# Autodesk Inventor assembly: embasev2
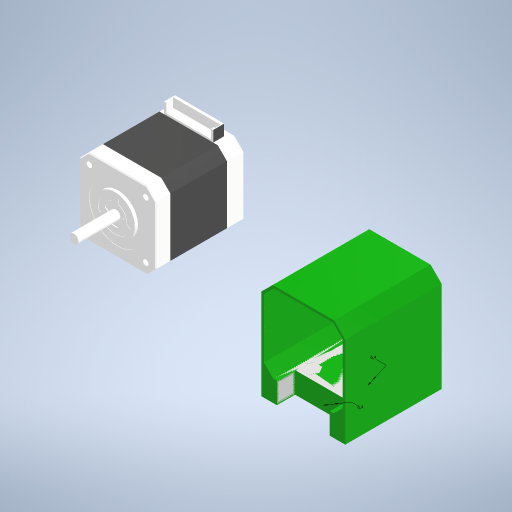
[picture p0: Inventor's stored thumbnail of the model, 512x512]
Saved by Autodesk Inventor 2024.2 (Build 282272000, 272)
## iProperties
Created: 2023-12-11
Part Number: embasev2
Document SubType Name: Assembly
Designer: adrie
Author: adrie
## Documents named in this file (4)
- C:\Users\adrie\Desktop\meca_robotbebou\embasev2\embasev2.iam
- C:\Users\adrie\Desktop\meca_robotbebou\SF2423-10B41_MIR1_MIR4.ipt
- C:\Users\adrie\Desktop\meca_robotbebou\support_moteurv3.ipt
- C:\Users\adrie\Desktop\meca_robotbebou\embasev2\support_moteur_v3.ipt
## Components (3 placed, 3 different names)
1. SF2423-10B41_MIR1_MIR4:1
2. support_moteurv3:1 — Mate:1
3. support_moteur_v3:1 — Mate:1
## Relationships (1: Mate 1)
- Mate:1: support_moteurv3:1 ↔ support_moteur_v3:1
